# Autodesk Inventor assembly: Interfas_1
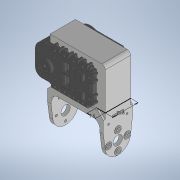
[picture p0: Inventor's stored thumbnail of the model, 180x180]
Saved by Autodesk Inventor 2021.3 (Build 253353000, 353)
## iProperties
Created: 2022-01-30
Part Number: Interfas_1
Document SubType Name: Assembly
Designer: epm01
Author: epm01
## Documents named in this file (3)
- D:\Archivos\2020-2\Papime\Banco_serial\Interfas_1.iam
- D:\Archivos\2020-2\Papime\Banco_serial\Bracket_bas.ipt
- D:\Archivos\2020-2\Papime\Banco_serial\AX-12A.iam
## Components (2 placed, 2 different names)
1. AX-12A:1 [sub-assembly] — Coincidencia:1, Coincidencia:2, Nivelación:1
2. Bracket_bas:1 — Coincidencia:1, Coincidencia:2, Nivelación:1
## Relationships (3: Mate 2, Flush 1)
- Coincidencia:1 [Mate]: AX-12A:1 ↔ Bracket_bas:1
- Coincidencia:2 [Mate]: AX-12A:1 ↔ Bracket_bas:1
- Nivelación:1 [Flush]: AX-12A:1 ↔ Bracket_bas:1
